# Autodesk Inventor assembly: Tuer_einheit_2
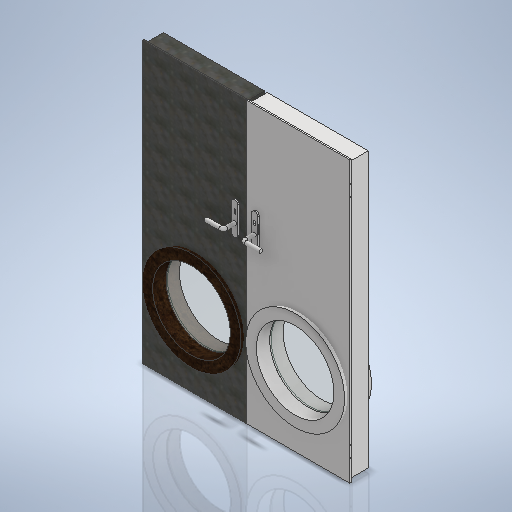
[picture p0: Inventor's stored thumbnail of the model, 512x512]
Saved by Autodesk Inventor 2025.1 (Build 291241000, 241)
## iProperties
Created: 2024-08-07
Part Number: Tuer_einheit_2
Document SubType Name: Assembly
Designer: ffogue
Author: ffogue
## Documents named in this file (3)
- C:\Users\ffogue\Documents\Inventor\BrandschutzTuer\Tuer_einheit_2.iam
- C:\Users\ffogue\Documents\Inventor\BrandschutzTuer\Tuer_MIR.iam
- C:\Users\ffogue\Documents\Inventor\BrandschutzTuer\Tuer.iam
## Components (2 placed, 2 different names)
1. Tuer_MIR:1 [sub-assembly] — Flush:1, Flush:2, Mate:1
2. Tuer:1 [sub-assembly] — Flush:1, Flush:2, Mate:1
## Relationships (3: Flush 2, Mate 1)
- Flush:1: Tuer_MIR:1 ↔ Tuer:1
- Flush:2: Tuer_MIR:1 ↔ Tuer:1
- Mate:1: Tuer_MIR:1 ↔ Tuer:1
